# Autodesk Inventor assembly: Arm
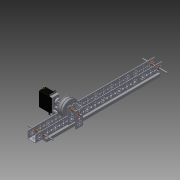
[picture p0: Inventor's stored thumbnail of the model, 180x180]
Saved by Autodesk Inventor 2014 SP2 (Build 180246200, 246)
## iProperties
Created: 2014-09-12
Part Number: Arm
Document SubType Name: Assembly
Designer: Allison
Author: Allison
## Documents named in this file (13)
- C:\Users\Allison\Documents\Inventor\InventorMasterProject\Arm.iam
- C:\Users\Allison\Documents\Inventor\InventorMasterProject\Tetrix\Channel\416mm Channel.ipt
- C:\Users\Allison\Documents\Inventor\InventorMasterProject\16 Drawer Slide.ipt
- C:\Users\Allison\Documents\Inventor\InventorMasterProject\Tetrix\Hubs and Axles\Bronze Bushing.ipt
- C:\Users\Allison\Documents\Inventor\InventorMasterProject\Tetrix\Hubs and Axles\Short Axle.ipt
- C:\Users\Allison\Documents\Inventor\InventorMasterProject\Tetrix\Hubs and Axles\Axle Hub.ipt
- C:\Users\Allison\Documents\Inventor\InventorMasterProject\Tetrix\Servos\Quarter Scale Servo.ipt
- C:\Users\Allison\Documents\Inventor\InventorMasterProject\Tetrix\Servos\Quarter-Scale Servo Front Mount Bracket.ipt
- C:\Users\Allison\Documents\Inventor\InventorMasterProject\Tetrix\Standoffs\1.25 Inch Standoff.ipt
- C:\Users\Allison\Documents\Inventor\InventorMasterProject\Tetrix\Servos\Servo Horn Metal.ipt
- C:\Users\Allison\Documents\Inventor\InventorMasterProject\Spool.ipt
- C:\Users\Allison\Documents\Inventor\InventorMasterProject\Servo Channel.ipt
- C:\Users\Allison\Documents\Inventor\InventorMasterProject\Tetrix\Channel\96mm Channel.ipt
## Components (23 placed, 12 different names)
1. 96mm Channel:1 — Insert:52, Insert:53, Flush:2, Flush:3, Mate:15
2. 416mm Channel:1 — Mate:1, Flush:1, Mate:2, Angle:1, Insert:39, Insert:40, Insert:41, Insert:42, Insert:51, Mate:14, Flush:2, Flush:3, Mate:15
3. 16 Drawer Slide:1 — Mate:1, Flush:1, Mate:3
4. Quarter Scale Servo:1 — Insert:22, Insert:23, Insert:28
5. Quarter-Scale Servo Front Mount Bracket:1 — Insert:22, Insert:23, Insert:24, Insert:26, Insert:27
6. 1.25 Inch Standoff:1 — Insert:24, Insert:39
7. 1.25 Inch Standoff:2 — Insert:26
8. 1.25 Inch Standoff:3 — Insert:27
9. 1.25 Inch Standoff:4 — Insert:40
10. Servo Horn Metal:1 — Insert:28, Insert:29, Insert:30
11. Axle Hub:3 — Insert:29, Insert:30, Insert:31
12. Short Axle:3 — Insert:31, Mate:5
13. Spool:1 — Insert:34
14. Axle Hub:4 — Insert:34, Mate:5
15. Servo Channel:1 — Insert:37, Insert:38, Insert:41, Insert:42
16. Bronze Bushing:6 — Insert:38
17. Bronze Bushing:7 — Insert:37
18. Bronze Bushing:16 — Insert:53
19. Short Axle:10 — Mate:13
20. Bronze Bushing:17 — Mate:13, Insert:52
21. Bronze Bushing:18 — Insert:51
22. Short Axle:11 — Mate:14
23. Bronze Bushing:19
## Relationships (30: Insert 19, Mate 7, Flush 3, Angle 1)
- Mate:1: 416mm Channel:1 ↔ 16 Drawer Slide:1
- Flush:1 (38.1 mm): 416mm Channel:1 ↔ 16 Drawer Slide:1
- Mate:2: 416mm Channel:1
- Angle:1 (0 deg): 416mm Channel:1
- Mate:3: 16 Drawer Slide:1
- Insert:22: Quarter Scale Servo:1 ↔ Quarter-Scale Servo Front Mount Bracket:1
- Insert:23: Quarter Scale Servo:1 ↔ Quarter-Scale Servo Front Mount Bracket:1
- Insert:24: Quarter-Scale Servo Front Mount Bracket:1 ↔ 1.25 Inch Standoff:1
- Insert:26: Quarter-Scale Servo Front Mount Bracket:1 ↔ 1.25 Inch Standoff:2
- Insert:27: Quarter-Scale Servo Front Mount Bracket:1 ↔ 1.25 Inch Standoff:3
- Insert:28: Quarter Scale Servo:1 ↔ Servo Horn Metal:1
- Insert:29: Servo Horn Metal:1 ↔ Axle Hub:3
- Insert:30: Servo Horn Metal:1 ↔ Axle Hub:3
- Insert:31: Axle Hub:3 ↔ Short Axle:3
- Insert:34: Spool:1 ↔ Axle Hub:4
- Mate:5: Short Axle:3 ↔ Axle Hub:4
- Insert:37: Servo Channel:1 ↔ Bronze Bushing:7
- Insert:38: Servo Channel:1 ↔ Bronze Bushing:6
- Insert:39: 416mm Channel:1 ↔ 1.25 Inch Standoff:1
- Insert:40: 416mm Channel:1 ↔ 1.25 Inch Standoff:4
- Insert:41: 416mm Channel:1 ↔ Servo Channel:1
- Insert:42: 416mm Channel:1 ↔ Servo Channel:1
- Mate:13: Short Axle:10 ↔ Bronze Bushing:17
- Insert:51: 416mm Channel:1 ↔ Bronze Bushing:18
- Mate:14: 416mm Channel:1 ↔ Short Axle:11
- Insert:52: 96mm Channel:1 ↔ Bronze Bushing:17
- Insert:53: 96mm Channel:1 ↔ Bronze Bushing:16
- Flush:2: 96mm Channel:1 ↔ 416mm Channel:1
- Flush:3: 96mm Channel:1 ↔ 416mm Channel:1
- Mate:15: 96mm Channel:1 ↔ 416mm Channel:1
